# Autodesk Inventor assembly: Vise_POS_REP
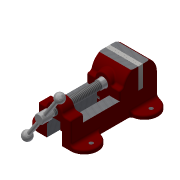
[picture p0: Inventor's stored thumbnail of the model, 180x180]
Saved by Autodesk Inventor 2022 (Build 260148000, 148)
## iProperties
Created: 2006-01-18
Part Number: Vise_POS_REP
Document SubType Name: Assembly
Designer: PMiller
Mass: 5339.96 g
Surface Area: 1407.98 cm^2
Volume: 680.25 cm^3
Density: 7.85 g/cm^3
Author: PMiller
## Documents named in this file (10)
- C:\Autodesk Inventor 2022 Advanced Assembly Modeling Practice Files\Vise_POS_REP_Assembly\Vise_POS_REP.iam
- C:\Autodesk Inventor 2022 Advanced Assembly Modeling Practice Files\Vise_POS_REP_Assembly\Base.ipt
- C:\Autodesk Inventor 2022 Advanced Assembly Modeling Practice Files\Vise_POS_REP_Assembly\Sliding_Jaw.ipt
- C:\Autodesk Inventor 2022 Advanced Assembly Modeling Practice Files\Vise_POS_REP_Assembly\Screw_Sub.iam
- C:\Autodesk Inventor 2022 Advanced Assembly Modeling Practice Files\Vise_POS_REP_Assembly\Collar.ipt
- C:\Autodesk Inventor 2022 Advanced Assembly Modeling Practice Files\Vise_POS_REP_Assembly\Jaw_Plate.ipt
- C:\Autodesk Inventor 2022 Advanced Assembly Modeling Practice Files\Vise_POS_REP_Assembly\Set_Screw.ipt
- C:\Autodesk Inventor 2022 Advanced Assembly Modeling Practice Files\Vise_POS_REP_Assembly\Slide_Key.ipt
- C:\Autodesk Inventor 2022 Advanced Assembly Modeling Practice Files\Vise_POS_REP_Assembly\Special_Key.ipt
- C:\Autodesk Inventor 2022 Advanced Assembly Modeling Practice Files\Vise_POS_REP_Assembly\1_4-0.75-UNC.ipt
## Components (15 placed, 9 different names)
1. Base:1 — Flush:1, Flush:2, Insert:1, Insert:2, Mate:2, Mate:4, Rotation/Translation:1
2. Sliding_Jaw:1 — Flush:1, Flush:2, Insert:3, Insert:4, Insert:11, Mate:1, Mate:3, Mate:5, Mate:6, Insert:12, Insert:13
3. Screw_Sub:1 [sub-assembly] — Insert:9, Insert:10, Rotation/Translation:1
4. Collar:1 — Insert:10, Insert:11
5. Jaw_Plate:1 — Insert:3, Insert:4, Insert:7, Insert:8, Mate:7
6. Jaw_Plate:2 — Insert:1, Insert:2, Insert:5, Insert:6, Mate:7
7. Set_Screw:1 — Insert:12
8. Set_Screw:2 — Insert:13
9. Slide_Key:1 — Mate:1, Mate:2, Mate:6
10. Slide_Key:2 — Mate:3, Mate:4, Mate:5
11. Special_Key:1 — Insert:9
12. Cross Recessed Flat Countersunk Head Machine Screw - Type I - Inch 1/4-20 x 3/4:1 — Insert:7
13. Cross Recessed Flat Countersunk Head Machine Screw - Type I - Inch 1/4-20 x 3/4:2 — Insert:8
14. Cross Recessed Flat Countersunk Head Machine Screw - Type I - Inch 1/4-20 x 3/4:3 — Insert:5
15. Cross Recessed Flat Countersunk Head Machine Screw - Type I - Inch 1/4-20 x 3/4:4 — Insert:6
## Relationships (23: Insert 13, Mate 7, Flush 2, RelateRotateTranslate 1)
- Flush:1: Base:1 ↔ Sliding_Jaw:1
- Flush:2: Base:1 ↔ Sliding_Jaw:1
- Insert:1: Base:1 ↔ Jaw_Plate:2
- Insert:2: Base:1 ↔ Jaw_Plate:2
- Insert:3: Sliding_Jaw:1 ↔ Jaw_Plate:1
- Insert:4: Sliding_Jaw:1 ↔ Jaw_Plate:1
- Insert:5: Jaw_Plate:2 ↔ Cross Recessed Flat Countersunk Head Machine Screw - Type I - Inch 1/4-20 x 3/4:3
- Insert:6: Jaw_Plate:2 ↔ Cross Recessed Flat Countersunk Head Machine Screw - Type I - Inch 1/4-20 x 3/4:4
- Insert:7: Jaw_Plate:1 ↔ Cross Recessed Flat Countersunk Head Machine Screw - Type I - Inch 1/4-20 x 3/4:1
- Insert:8: Jaw_Plate:1 ↔ Cross Recessed Flat Countersunk Head Machine Screw - Type I - Inch 1/4-20 x 3/4:2
- Insert:9: Screw_Sub:1 ↔ Special_Key:1
- Insert:10: Screw_Sub:1 ↔ Collar:1
- Insert:11 (-11.1125 mm): Sliding_Jaw:1 ↔ Collar:1
- Mate:1: Sliding_Jaw:1 ↔ Slide_Key:1
- Mate:2: Base:1 ↔ Slide_Key:1
- Mate:3: Sliding_Jaw:1 ↔ Slide_Key:2
- Mate:4: Base:1 ↔ Slide_Key:2
- Mate:5: Sliding_Jaw:1 ↔ Slide_Key:2
- Mate:6: Sliding_Jaw:1 ↔ Slide_Key:1
- Insert:12: Sliding_Jaw:1 ↔ Set_Screw:1
- Insert:13: Sliding_Jaw:1 ↔ Set_Screw:2
- Rotation/Translation:1 [RelateRotateTranslate] (3.81 mm): Base:1 ↔ Screw_Sub:1
- Mate:7: Jaw_Plate:1 ↔ Jaw_Plate:2
